# Autodesk Inventor assembly: EscritorioV4
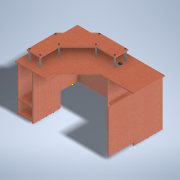
[picture p0: Inventor's stored thumbnail of the model, 180x180]
Saved by Autodesk Inventor 2020.3 (Build 243373000, 373)
## iProperties
Created: 2020-12-15
Part Number: EscritorioV4
Document SubType Name: Assembly
Designer: codig
Author: codig
## Documents named in this file (18)
- C:\Users\codig\OneDrive\Documentos\GrabCAD\EscritorioV4\EscritorioV4.iam
- C:\Users\codig\OneDrive\Documentos\GrabCAD\EscritorioV4\BaseCajoneras.ipt
- C:\Users\codig\OneDrive\Documentos\GrabCAD\EscritorioV4\BasePC.ipt
- C:\Users\codig\OneDrive\Documentos\GrabCAD\EscritorioV4\FondoMuralla.ipt
- C:\Users\codig\OneDrive\Documentos\GrabCAD\EscritorioV4\LateralInteriorCajoneras.ipt
- C:\Users\codig\OneDrive\Documentos\GrabCAD\EscritorioV4\LateralInteriorPC.ipt
- C:\Users\codig\OneDrive\Documentos\GrabCAD\EscritorioV4\LateralMayor.ipt
- C:\Users\codig\OneDrive\Documentos\GrabCAD\EscritorioV4\LateralMenor.ipt
- C:\Users\codig\OneDrive\Documentos\GrabCAD\EscritorioV4\puerta.ipt
- C:\Users\codig\OneDrive\Documentos\GrabCAD\EscritorioV4\repisa.ipt
- C:\Users\codig\OneDrive\Documentos\GrabCAD\EscritorioV4\Tapa01.ipt
- C:\Users\codig\OneDrive\Documentos\GrabCAD\EscritorioV4\Tapa02.ipt
- C:\Users\codig\OneDrive\Documentos\GrabCAD\EscritorioV4\TarugoRepisa.ipt
- C:\Users\codig\OneDrive\Documentos\GrabCAD\EscritorioV4\Tarugos.ipt
- C:\Users\codig\OneDrive\Documentos\GrabCAD\EscritorioV4\SoporteAluminio\Pieza1.ipt
- C:\Users\codig\OneDrive\Documentos\GrabCAD\EscritorioV4\SoporteAluminio\Pieza3.ipt
- C:\Users\codig\OneDrive\Documentos\GrabCAD\EscritorioV4\PataMesa\PataMesa.iam
- C:\Users\codig\OneDrive\Documentos\GrabCAD\EscritorioV4\Bosquejo Pasacables\pasacables.iam
## Components (94 placed, 17 different names)
1. BaseCajoneras:1 — Insertar:84, Insertar:85, Insertar:86, Insertar:87, Insertar:88, Insertar:89
2. BasePC:1 — Insertar:49, Insertar:50, Insertar:53, Insertar:54, Insertar:55, Insertar:56
3. BasePC:2 — Insertar:43, Insertar:44, Insertar:45, Insertar:46, Insertar:47, Insertar:48
4. FondoMuralla:1 — Insertar:16, Insertar:17, Insertar:18, Insertar:25, Insertar:26, Insertar:27, Insertar:57, Insertar:58, Insertar:59, Insertar:66, Insertar:67, Insertar:68, Coincidencia:2, Insertar:135, Insertar:136, Insertar:137, Insertar:138
5. LateralInteriorCajoneras:1 — Insertar:69, Insertar:70, Insertar:71, Insertar:72, Insertar:73, Insertar:74, Insertar:75, Insertar:76, Insertar:77, Insertar:81, Insertar:82, Insertar:83, Insertar:93, Insertar:94, Insertar:95, Insertar:132, Insertar:133, Insertar:134
6. LateralInteriorPC:1 — Insertar:34, Insertar:35, Insertar:36, Insertar:37, Insertar:38, Insertar:39, Insertar:40, Insertar:41, Insertar:42, Insertar:51, Insertar:52, Insertar:126, Insertar:127, Insertar:128
7. LateralMayor:1 — Insertar:19, Insertar:20, Insertar:21, Insertar:22, Insertar:23, Insertar:24, Insertar:28, Insertar:29, Insertar:30, Insertar:31, Insertar:32, Insertar:33, Insertar:123, Insertar:124, Insertar:125
8. LateralMenor:1 — Insertar:60, Insertar:61, Insertar:62, Insertar:63, Insertar:64, Insertar:65, Insertar:78, Insertar:79, Insertar:80, Insertar:90, Insertar:91, Insertar:92, Coincidencia:1, Coincidencia:3, Coincidencia:5, Insertar:129, Insertar:130, Insertar:131
9. puerta:1 — Coincidencia:3, Coincidencia:4, Coincidencia:5
10. repisa:1 — Tangente:1, Coincidencia:1, Coincidencia:2
11. Tapa01:1 — Insertar:1, Insertar:2, Insertar:3, Insertar:4, Insertar:5, Insertar:6, Insertar:7, Insertar:8, Insertar:9, Insertar:10, Insertar:11, Insertar:12, Insertar:13, Insertar:14, Insertar:15, Coincidencia:4, Insertar:96, Insertar:97, Insertar:98, Insertar:99, Insertar:100, Insertar:101, Insertar:102, Insertar:103, Insertar:139, Insertar:140
12. TarugoRepisa:1 — Insertar:90
13. Tarugos:1 — Insertar:2, Insertar:22
14. Tarugos:2 — Insertar:1, Insertar:24
15. Tarugos:3 — Insertar:5, Insertar:16
16. Tarugos:4 — Insertar:6, Insertar:35
17. Tarugos:5 — Insertar:3, Insertar:23
18. Tarugos:6 — Insertar:4, Insertar:18
19. Tarugos:7 — Insertar:28, Insertar:48
20. Tarugos:8 — Insertar:15, Insertar:36
21. Tarugos:9 — Insertar:32, Insertar:49
22. Tarugos:10 — Insertar:42, Insertar:54
23. Tarugos:11 — Insertar:41, Insertar:55
24. Tarugos:12 — Insertar:37, Insertar:44
25. Tarugos:13 — Insertar:30, Insertar:46
26. Tarugos:14 — Insertar:21, Insertar:27
27. Tarugos:15 — Insertar:19, Insertar:25
28. Tarugos:16 — Insertar:10, Insertar:17
29. Tarugos:17 — Insertar:12, Insertar:60
30. Tarugos:18 — Insertar:14, Insertar:34
31. Tarugos:19 — Insertar:33, Insertar:53
32. Tarugos:20 — Insertar:39, Insertar:45, Insertar:52
33. Tarugos:21 — Insertar:38, Insertar:43, Insertar:51
34. Tarugos:22 — Insertar:58, Insertar:61
35. Tarugos:23 — Insertar:57, Insertar:64
36. Tarugos:24 — Insertar:31, Insertar:50
37. Tarugos:25 — Insertar:29, Insertar:47
38. Tarugos:26 — Insertar:20, Insertar:26
39. Tarugos:27 — Insertar:9, Insertar:69, Insertar:76
40. Tarugos:28 — Insertar:8, Insertar:75
41. Tarugos:29 — Insertar:7, Insertar:74, Insertar:77
42. Tarugos:30 — Insertar:11, Insertar:62
43. Tarugos:31 — Insertar:13, Insertar:63
44. Tarugos:32 — Insertar:40, Insertar:56
45. Tarugos:33 — Insertar:59, Insertar:65
46. Tarugos:34 — Insertar:67, Insertar:72
47. Tarugos:35 — Insertar:66, Insertar:73
48. Tarugos:36 — Insertar:68, Insertar:70, Insertar:71
49. Tarugos:37 — Insertar:78, Insertar:87
50. Tarugos:38 — Insertar:82, Insertar:88
51. Tarugos:39 — Insertar:83, Insertar:84
52. Tarugos:40 — Insertar:79, Insertar:86
53. Tarugos:41 — Insertar:80, Insertar:85
54. Tarugos:42 — Insertar:81, Insertar:89
55. TarugoRepisa:2 — Insertar:92
56. TarugoRepisa:3 — Insertar:91, Tangente:1
57. TarugoRepisa:4 — Insertar:94
58. TarugoRepisa:5 — Insertar:93
59. TarugoRepisa:6 — Insertar:95
60. Pieza1:1 — Insertar:96, Insertar:141
61. Pieza1:2 — Insertar:97, Insertar:142
62. Pieza1:3 — Insertar:98, Insertar:143
63. Pieza1:4 — Insertar:101, Insertar:146
64. Pieza1:5 — Insertar:100, Insertar:145
65. Pieza1:6 — Insertar:99, Insertar:144
66. Pieza1:7 — Insertar:103, Insertar:148
67. Pieza1:8 — Insertar:102, Insertar:147
68. PataMesa:1 [sub-assembly] — Insertar:128
69. PataMesa:2 [sub-assembly] — Insertar:127
70. PataMesa:3 [sub-assembly] — Insertar:126
71. PataMesa:4 [sub-assembly] — Insertar:125
72. PataMesa:5 [sub-assembly] — Insertar:124
73. PataMesa:6 [sub-assembly] — Insertar:123
74. PataMesa:7 [sub-assembly] — Insertar:134
75. PataMesa:8 [sub-assembly] — Insertar:133
76. PataMesa:9 [sub-assembly] — Insertar:132
77. PataMesa:10 [sub-assembly] — Insertar:131
78. PataMesa:11 [sub-assembly] — Insertar:130
79. PataMesa:12 [sub-assembly] — Insertar:129
80. PataMesa:13 [sub-assembly] — Insertar:135
81. PataMesa:14 [sub-assembly] — Insertar:136
82. PataMesa:15 [sub-assembly] — Insertar:137
83. pasacables:1 [sub-assembly] — Insertar:138
84. pasacables:2 [sub-assembly] — Insertar:140
85. pasacables:3 [sub-assembly] — Insertar:139
86. Tapa02:1 — Insertar:141, Insertar:142, Insertar:143, Insertar:144, Insertar:145, Insertar:146, Insertar:147, Insertar:148, Insertar:149, Insertar:150, Insertar:151, Insertar:152, Insertar:153, Insertar:154, Insertar:155, Insertar:156
87. Pieza3:1 — Insertar:149
88. Pieza3:2 — Insertar:150
89. Pieza3:3 — Insertar:151
90. Pieza3:4 — Insertar:152
91. Pieza3:5 — Insertar:153
92. Pieza3:6 — Insertar:156
93. Pieza3:7 — Insertar:155
94. Pieza3:8 — Insertar:154
## Relationships (143: Insert 137, Mate 5, Tangent 1)
- Insertar:1: Tapa01:1 ↔ Tarugos:2
- Insertar:2: Tapa01:1 ↔ Tarugos:1
- Insertar:3: Tapa01:1 ↔ Tarugos:5
- Insertar:4: Tapa01:1 ↔ Tarugos:6
- Insertar:5: Tapa01:1 ↔ Tarugos:3
- Insertar:6: Tapa01:1 ↔ Tarugos:4
- Insertar:7: Tapa01:1 ↔ Tarugos:29
- Insertar:8: Tapa01:1 ↔ Tarugos:28
- Insertar:9: Tapa01:1 ↔ Tarugos:27
- Insertar:10: Tapa01:1 ↔ Tarugos:16
- Insertar:11: Tapa01:1 ↔ Tarugos:30
- Insertar:12: Tapa01:1 ↔ Tarugos:17
- Insertar:13: Tapa01:1 ↔ Tarugos:31
- Insertar:14: Tapa01:1 ↔ Tarugos:18
- Insertar:15: Tapa01:1 ↔ Tarugos:8
- Insertar:16: FondoMuralla:1 ↔ Tarugos:3
- Insertar:17: FondoMuralla:1 ↔ Tarugos:16
- Insertar:18: FondoMuralla:1 ↔ Tarugos:6
- Insertar:19: LateralMayor:1 ↔ Tarugos:15
- Insertar:20: LateralMayor:1 ↔ Tarugos:26
- Insertar:21: LateralMayor:1 ↔ Tarugos:14
- Insertar:22: LateralMayor:1 ↔ Tarugos:1
- Insertar:23: LateralMayor:1 ↔ Tarugos:5
- Insertar:24: LateralMayor:1 ↔ Tarugos:2
- Insertar:25: FondoMuralla:1 ↔ Tarugos:15
- Insertar:26: FondoMuralla:1 ↔ Tarugos:26
- Insertar:27: FondoMuralla:1 ↔ Tarugos:14
- Insertar:28: LateralMayor:1 ↔ Tarugos:7
- Insertar:29: LateralMayor:1 ↔ Tarugos:25
- Insertar:30: LateralMayor:1 ↔ Tarugos:13
- Insertar:31: LateralMayor:1 ↔ Tarugos:24
- Insertar:32: LateralMayor:1 ↔ Tarugos:9
- Insertar:33: LateralMayor:1 ↔ Tarugos:19
- Insertar:34: LateralInteriorPC:1 ↔ Tarugos:18
- Insertar:35: LateralInteriorPC:1 ↔ Tarugos:4
- Insertar:36: LateralInteriorPC:1 ↔ Tarugos:8
- Insertar:37: LateralInteriorPC:1 ↔ Tarugos:12
- Insertar:38: LateralInteriorPC:1 ↔ Tarugos:21
- Insertar:39: LateralInteriorPC:1 ↔ Tarugos:20
- Insertar:40: LateralInteriorPC:1 ↔ Tarugos:32
- Insertar:41: LateralInteriorPC:1 ↔ Tarugos:11
- Insertar:42: LateralInteriorPC:1 ↔ Tarugos:10
- Insertar:43: BasePC:2 ↔ Tarugos:21
- Insertar:44: BasePC:2 ↔ Tarugos:12
- Insertar:45: BasePC:2 ↔ Tarugos:20
- Insertar:46: BasePC:2 ↔ Tarugos:13
- Insertar:47: BasePC:2 ↔ Tarugos:25
- Insertar:48: BasePC:2 ↔ Tarugos:7
- Insertar:49: BasePC:1 ↔ Tarugos:9
- Insertar:50: BasePC:1 ↔ Tarugos:24
- Insertar:51: LateralInteriorPC:1 ↔ Tarugos:21
- Insertar:52: LateralInteriorPC:1 ↔ Tarugos:20
- Insertar:53: BasePC:1 ↔ Tarugos:19
- Insertar:54: BasePC:1 ↔ Tarugos:10
- Insertar:55: BasePC:1 ↔ Tarugos:11
- Insertar:56: BasePC:1 ↔ Tarugos:32
- Insertar:57: FondoMuralla:1 ↔ Tarugos:23
- Insertar:58: FondoMuralla:1 ↔ Tarugos:22
- Insertar:59: FondoMuralla:1 ↔ Tarugos:33
- Insertar:60: LateralMenor:1 ↔ Tarugos:17
- Insertar:61: LateralMenor:1 ↔ Tarugos:22
- Insertar:62: LateralMenor:1 ↔ Tarugos:30
- Insertar:63: LateralMenor:1 ↔ Tarugos:31
- Insertar:64: LateralMenor:1 ↔ Tarugos:23
- Insertar:65: LateralMenor:1 ↔ Tarugos:33
- Insertar:66: FondoMuralla:1 ↔ Tarugos:35
- Insertar:67: FondoMuralla:1 ↔ Tarugos:34
- Insertar:68: FondoMuralla:1 ↔ Tarugos:36
- Insertar:69: LateralInteriorCajoneras:1 ↔ Tarugos:27
- Insertar:70: LateralInteriorCajoneras:1 ↔ Tarugos:36
- Insertar:71: LateralInteriorCajoneras:1 ↔ Tarugos:36
- Insertar:72: LateralInteriorCajoneras:1 ↔ Tarugos:34
- Insertar:73: LateralInteriorCajoneras:1 ↔ Tarugos:35
- Insertar:74: LateralInteriorCajoneras:1 ↔ Tarugos:29
- Insertar:75: LateralInteriorCajoneras:1 ↔ Tarugos:28
- Insertar:76: LateralInteriorCajoneras:1 ↔ Tarugos:27
- Insertar:77: LateralInteriorCajoneras:1 ↔ Tarugos:29
- Insertar:78: LateralMenor:1 ↔ Tarugos:37
- Insertar:79: LateralMenor:1 ↔ Tarugos:40
- Insertar:80: LateralMenor:1 ↔ Tarugos:41
- Insertar:81: LateralInteriorCajoneras:1 ↔ Tarugos:42
- Insertar:82: LateralInteriorCajoneras:1 ↔ Tarugos:38
- Insertar:83: LateralInteriorCajoneras:1 ↔ Tarugos:39
- Insertar:84: BaseCajoneras:1 ↔ Tarugos:39
- Insertar:85: BaseCajoneras:1 ↔ Tarugos:41
- Insertar:86: BaseCajoneras:1 ↔ Tarugos:40
- Insertar:87: BaseCajoneras:1 ↔ Tarugos:37
- Insertar:88: BaseCajoneras:1 ↔ Tarugos:38
- Insertar:89: BaseCajoneras:1 ↔ Tarugos:42
- Insertar:90: LateralMenor:1 ↔ TarugoRepisa:1
- Insertar:91: LateralMenor:1 ↔ TarugoRepisa:3
- Insertar:92: LateralMenor:1 ↔ TarugoRepisa:2
- Insertar:93: LateralInteriorCajoneras:1 ↔ TarugoRepisa:5
- Insertar:94: LateralInteriorCajoneras:1 ↔ TarugoRepisa:4
- Insertar:95: LateralInteriorCajoneras:1 ↔ TarugoRepisa:6
- Tangente:1: repisa:1 ↔ TarugoRepisa:3
- Coincidencia:1 [Mate]: LateralMenor:1 ↔ repisa:1
- Coincidencia:2 [Mate]: FondoMuralla:1 ↔ repisa:1
- Coincidencia:3 [Mate]: LateralMenor:1 ↔ puerta:1
- Coincidencia:4 [Mate]: puerta:1 ↔ Tapa01:1
- Coincidencia:5 [Mate]: LateralMenor:1 ↔ puerta:1
- Insertar:96: Tapa01:1 ↔ Pieza1:1
- Insertar:97: Tapa01:1 ↔ Pieza1:2
- Insertar:98: Tapa01:1 ↔ Pieza1:3
- Insertar:99: Tapa01:1 ↔ Pieza1:6
- Insertar:100: Tapa01:1 ↔ Pieza1:5
- Insertar:101: Tapa01:1 ↔ Pieza1:4
- Insertar:102: Tapa01:1 ↔ Pieza1:8
- Insertar:103: Tapa01:1 ↔ Pieza1:7
- Insertar:123: LateralMayor:1 ↔ PataMesa:6
- Insertar:124: LateralMayor:1 ↔ PataMesa:5
- Insertar:125: LateralMayor:1 ↔ PataMesa:4
- Insertar:126: LateralInteriorPC:1 ↔ PataMesa:3
- Insertar:127: LateralInteriorPC:1 ↔ PataMesa:2
- Insertar:128: LateralInteriorPC:1 ↔ PataMesa:1
- Insertar:129: LateralMenor:1 ↔ PataMesa:12
- Insertar:130: LateralMenor:1 ↔ PataMesa:11
- Insertar:131: LateralMenor:1 ↔ PataMesa:10
- Insertar:132: LateralInteriorCajoneras:1 ↔ PataMesa:9
- Insertar:133: LateralInteriorCajoneras:1 ↔ PataMesa:8
- Insertar:134: LateralInteriorCajoneras:1 ↔ PataMesa:7
- Insertar:135: FondoMuralla:1 ↔ PataMesa:13
- Insertar:136: FondoMuralla:1 ↔ PataMesa:14
- Insertar:137: FondoMuralla:1 ↔ PataMesa:15
- Insertar:138: FondoMuralla:1 ↔ pasacables:1
- Insertar:139: Tapa01:1 ↔ pasacables:3
- Insertar:140: Tapa01:1 ↔ pasacables:2
- Insertar:141: Pieza1:1 ↔ Tapa02:1
- Insertar:142: Pieza1:2 ↔ Tapa02:1
- Insertar:143: Pieza1:3 ↔ Tapa02:1
- Insertar:144: Pieza1:6 ↔ Tapa02:1
- Insertar:145: Pieza1:5 ↔ Tapa02:1
- Insertar:146: Pieza1:4 ↔ Tapa02:1
- Insertar:147: Pieza1:8 ↔ Tapa02:1
- Insertar:148: Pieza1:7 ↔ Tapa02:1
- Insertar:149: Tapa02:1 ↔ Pieza3:1
- Insertar:150: Tapa02:1 ↔ Pieza3:2
- Insertar:151: Tapa02:1 ↔ Pieza3:3
- Insertar:152: Tapa02:1 ↔ Pieza3:4
- Insertar:153: Tapa02:1 ↔ Pieza3:5
- Insertar:154: Tapa02:1 ↔ Pieza3:8
- Insertar:155: Tapa02:1 ↔ Pieza3:7
- Insertar:156: Tapa02:1 ↔ Pieza3:6
